# Autodesk Inventor assembly: steeringarm.ipt
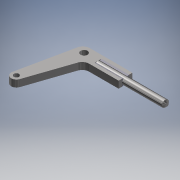
[picture p0: Inventor's stored thumbnail of the model, 180x180]
Saved by Autodesk Inventor 2018 (Build 220112000, 112)
## iProperties
Created: 2018-08-06
Part Number: steeringarm.ipt
Document SubType Name: Weldment
Designer: Cole Tucker
Weld Material: Welded Aluminum-6061
Mass: 301.448 g
Surface Area: 174.752 cm^2
Volume: 39.2487 cm^3
Density: 7.68045 g/cm^3
Author: Cole Tucker
## Documents named in this file (3)
- C:\Users\Cole Tucker\OneDrive\FRC-mxpProject\Cad\chassis\Inventor\v2\steeringarm.iam
- C:\Users\Cole Tucker\OneDrive\FRC-mxpProject\Cad\chassis\Inventor\v2\steeringarm.ipt
- C:\Users\Cole Tucker\OneDrive\FRC-mxpProject\Cad\chassis\Inventor\v2\frontshaft.ipt
## Components (2 placed, 2 different names)
1. steeringarm:1 — Mate:1, Mate:2, Mate:3
2. Shaft:1 — Mate:1, Mate:2, Mate:3
## Relationships (3: Mate 3)
- Mate:1 (6.35 mm): steeringarm:1 ↔ Shaft:1
- Mate:2: steeringarm:1 ↔ Shaft:1
- Mate:3 (-6.35 mm): steeringarm:1 ↔ Shaft:1
